# Autodesk Inventor assembly: Assembly7
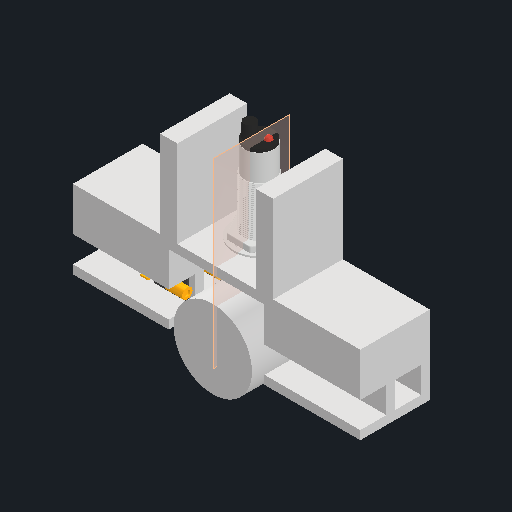
[picture p0: Inventor's stored thumbnail of the model, 512x512]
Saved by Autodesk Inventor 2027.1 (Build 311270010, 270A)
## iProperties
Created: 2026-09-29
Part Number: Assembly7
Document SubType Name: Assembly
Designer: daniel
Author: daniel
## Documents named in this file (5)
- E:\Apps\AutodeskInventor\University\MCT333_Design_of_Mechatronics_Systems_1\CAD\FEED and Sorting\Assembly7.iam
- E:\Apps\AutodeskInventor\University\MCT333_Design_of_Mechatronics_Systems_1\CAD\FEED and Sorting\Part56.ipt
- E:\Apps\AutodeskInventor\University\MCT333_Design_of_Mechatronics_Systems_1\CAD\off_the_shelf_components\18mm-inductive-proximity-sensor-taiss-4\Inductive Proximity Sensor Assembly\Inductive Proximity Sensor Assembly.iam
- E:\Apps\AutodeskInventor\University\MCT333_Design_of_Mechatronics_Systems_1\CAD\FEED and Sorting\Part23.ipt
- E:\Apps\AutodeskInventor\University\MCT333_Design_of_Mechatronics_Systems_1\CAD\off_the_shelf_components\LaserModule\LaserModule.ipt
## Components (5 placed, 4 different names)
1. Part56:1 — Mate:1, Mate:4, Mate:5, Mate:6, Flush:1, Flush:2, Mate:7, Mate:8, Flush:3
2. Inductive Proximity Sensor Assembly:1 [sub-assembly] — Mate:1, Mate:4, Tangent:1
3. LaserModule:1 — Mate:6, Flush:2, Mate:8
4. LaserModule:2 — Mate:5, Flush:1, Mate:7
5. Part23:1 — Flush:3, Tangent:1
## Relationships (10: Mate 6, Flush 3, Tangent 1)
- Mate:1: Part56:1 ↔ Inductive Proximity Sensor Assembly:1
- Mate:4: Part56:1 ↔ Inductive Proximity Sensor Assembly:1
- Mate:5: Part56:1 ↔ LaserModule:2
- Mate:6: Part56:1 ↔ LaserModule:1
- Flush:1: Part56:1 ↔ LaserModule:2
- Flush:2: Part56:1 ↔ LaserModule:1
- Mate:7: Part56:1 ↔ LaserModule:2
- Mate:8: Part56:1 ↔ LaserModule:1
- Flush:3: Part56:1 ↔ Part23:1
- Tangent:1: Inductive Proximity Sensor Assembly:1 ↔ Part23:1
